# Autodesk Inventor assembly: DuoCopter - Montagem
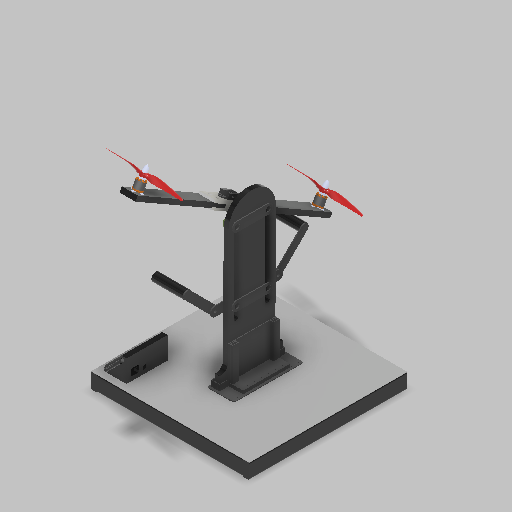
[picture p0: Inventor's stored thumbnail of the model, 512x512]
Saved by Autodesk Inventor 2025.2 (Build 292293000, 293)
## iProperties
Created: 2024-04-26
Part Number: DuoCopter - Montagem
Document SubType Name: Assembly
Designer: phmca
Author: phmca
## Documents named in this file (19)
- C:\Users\phmca\OneDrive\Área de Trabalho\GitHub\Modelos 3D\Montagem da planta\DuoCopter - Montagem.iam
- C:\Users\phmca\OneDrive\Área de Trabalho\GitHub\Modelos 3D\Montagem da planta\Chapa - aço galvanizado.ipt
- C:\Users\phmca\OneDrive\Área de Trabalho\GitHub\Modelos 3D\Montagem da planta\Painel Vertical.ipt
- C:\Users\phmca\OneDrive\Área de Trabalho\GitHub\Modelos 3D\Montagem da planta\Ripas - Base - 458 mm.ipt
- C:\Users\phmca\OneDrive\Área de Trabalho\GitHub\Modelos 3D\Montagem da planta\Ripas - Base - 500 mm.ipt
- C:\Users\phmca\OneDrive\Área de Trabalho\GitHub\Modelos 3D\Montagem da planta\Ripas - Base - 200 mm.ipt
- C:\Users\phmca\OneDrive\Área de Trabalho\GitHub\Modelos 3D\Montagem da planta\Modelos externos\Mancal de rolamento - SKF\SKF_UCFL 205.iam
- C:\Users\phmca\OneDrive\Área de Trabalho\GitHub\Modelos 3D\Montagem da planta\Junta.ipt
- C:\Users\phmca\OneDrive\Área de Trabalho\GitHub\Modelos 3D\Montagem da planta\Pás - Hastes.ipt
- C:\Users\phmca\OneDrive\Área de Trabalho\GitHub\Modelos 3D\Montagem da planta\Chapa - Aperto fixação.ipt
- C:\Users\phmca\OneDrive\Área de Trabalho\GitHub\Modelos 3D\Montagem da planta\Base - Batentes.ipt
- C:\Users\phmca\OneDrive\Área de Trabalho\GitHub\Modelos 3D\Montagem da planta\Batente limitador.ipt
- C:\Users\phmca\OneDrive\Área de Trabalho\GitHub\Modelos 3D\Montagem da planta\Base - Painel vertical.ipt
- C:\Users\phmca\OneDrive\Área de Trabalho\GitHub\Modelos 3D\Montagem da planta\Modelos externos\Motor brushless e hélices\assembly\assembly_motor.iam
- C:\Users\phmca\OneDrive\Área de Trabalho\GitHub\Modelos 3D\Montagem da planta\Case - IMU.ipt
- C:\Users\phmca\OneDrive\Área de Trabalho\GitHub\Modelos 3D\Montagem da planta\Modelos externos\Módulo MPU 6050\MPU_6050 v1.iam
- C:\Users\phmca\OneDrive\Área de Trabalho\CASE - IHM V2.ipt
- C:\Users\phmca\Downloads\nextion-3-5-hmi-nx4832t035-1.snapshot.7\Nextion 3.5 inch HMI (NX4832T035)\Nextion_3.5_HMI_NX4832T035\Nextion_3.5_HMI_NX4832T035\Nextion_3.5_HMI_NX4832T035.ipt
- C:\Users\phmca\OneDrive\Área de Trabalho\GitHub\Modelos 3D\Montagem da planta\Caneta - IHM.ipt
## Components (28 placed, 18 different names)
1. Chapa - aço galvanizado:1 — Alinhado:14, Alinhado:15, Coincidente:7, Coincidente:26, Coincidente:60, Coincidente:63
2. Painel Vertical:1 — Alinhado:9, Coincidente:3, Coincidente:5, Alinhado:13, Rotativa:1, Rotativa:2, Rotativa:4, Coincidente:13, Coincidente:16, Coincidente:27, Coincidente:31, Coincidente:36, Coincidente:37, Coincidente:46, Coincidente:61, Coincidente:62
3. Ripas - Base - 458 mm:1 — Rígida:3, Alinhado:15
4. Ripas - Base - 500 mm:1 — Rígida:2, Rígida:3, Coincidente:1, Coincidente:2
5. Ripas - Base - 500 mm:2 — Rígida:1, Alinhado:3, Alinhado:6, Alinhado:14, Coincidente:7
6. Ripas - Base - 458 mm:2 — Rígida:1, Rígida:2
7. Ripas - Base - 458 mm:3 — Alinhado:3, Coincidente:1
8. Ripas - Base - 458 mm:4 — Alinhado:6, Coincidente:2, Alinhado:9, Coincidente:3, Coincidente:4, Alinhado:11
9. Ripas - Base - 200 mm:1 — Alinhado:13
10. Ripas - Base - 200 mm:2 — Coincidente:4, Alinhado:11, Coincidente:5
11. SKF_UCFL 205:1 [sub-assembly] — Rotativa:1, Rotativa:2, Rotativa:3
12. Junta:1 — Rotativa:3, Coincidente:8, Coincidente:9, Alinhado:16, Coincidente:10, Coincidente:11, Alinhado:17, Rotativa:7, Alinhado:21
13. Pás - Hastes:1 — Coincidente:10, Coincidente:11, Alinhado:17, Coincidente:49, Tangente:1, Tangente:2
14. Pás - Hastes:2 — Coincidente:8, Coincidente:9, Alinhado:16, Coincidente:54
15. Chapa - Aperto fixação:1 — Rotativa:4, Coincidente:31
16. Base - Batentes:1 — Coincidente:13, Rotativa:5, Rotativa:6, Rotativa:8
17. Batente limitador:1 — Rotativa:5, Tangente:1, Rotativa:8, Tangente:2
18. Batente limitador:2 — Rotativa:6
19. Chapa - Aperto fixação:2 — Coincidente:16
20. Base - Painel vertical:1 — Coincidente:26, Coincidente:27, Coincidente:36, Coincidente:37, Coincidente:46
21. assembly_motor:1 [sub-assembly] — Coincidente:49
22. assembly_motor:2 [sub-assembly] — Coincidente:54
23. Case - IMU:1 — Rotativa:7, Alinhado:21, Rotativa:9
24. MPU_6050 v1:1 [sub-assembly] — Rotativa:9
25. Base - Painel vertical:3 — Coincidente:60, Coincidente:61, Coincidente:62
26. CASE - IHM V2:1 — Coincidente:63, Rotativa:10, Rotativa:11
27. Nextion_3.5_HMI_NX4832T035:1 — Rotativa:10
28. Caneta - IHM:1 — Rotativa:11
## Relationships (50: Mate 24, RevoluteJoint 11, Flush 10, WeldJoint 3, Tangent 2)
- Rígida:1 [WeldJoint]: Ripas - Base - 500 mm:2 ↔ Ripas - Base - 458 mm:2
- Rígida:2 [WeldJoint]: Ripas - Base - 500 mm:1 ↔ Ripas - Base - 458 mm:2
- Rígida:3 [WeldJoint]: Ripas - Base - 458 mm:1 ↔ Ripas - Base - 500 mm:1
- Alinhado:3 [Flush]: Ripas - Base - 500 mm:2 ↔ Ripas - Base - 458 mm:3
- Coincidente:1 [Mate]: Ripas - Base - 500 mm:1 ↔ Ripas - Base - 458 mm:3
- Alinhado:6 [Flush]: Ripas - Base - 500 mm:2 ↔ Ripas - Base - 458 mm:4
- Coincidente:2 [Mate]: Ripas - Base - 500 mm:1 ↔ Ripas - Base - 458 mm:4
- Alinhado:9 [Flush]: Painel Vertical:1 ↔ Ripas - Base - 458 mm:4
- Coincidente:3 [Mate]: Painel Vertical:1 ↔ Ripas - Base - 458 mm:4
- Coincidente:4 [Mate]: Ripas - Base - 458 mm:4 ↔ Ripas - Base - 200 mm:2
- Alinhado:11 [Flush]: Ripas - Base - 458 mm:4 ↔ Ripas - Base - 200 mm:2
- Coincidente:5 [Mate]: Painel Vertical:1 ↔ Ripas - Base - 200 mm:2
- Alinhado:13 [Flush]: Painel Vertical:1 ↔ Ripas - Base - 200 mm:1
- Alinhado:14 [Flush]: Chapa - aço galvanizado:1 ↔ Ripas - Base - 500 mm:2
- Alinhado:15 [Flush]: Chapa - aço galvanizado:1 ↔ Ripas - Base - 458 mm:1
- Coincidente:7 [Mate]: Chapa - aço galvanizado:1 ↔ Ripas - Base - 500 mm:2
- Rotativa:1 [RevoluteJoint]: Painel Vertical:1 ↔ SKF_UCFL 205:1
- Rotativa:2 [RevoluteJoint]: Painel Vertical:1 ↔ SKF_UCFL 205:1
- Rotativa:3 [RevoluteJoint]: SKF_UCFL 205:1 ↔ Junta:1
- Coincidente:8 [Mate]: Junta:1 ↔ Pás - Hastes:2
- Coincidente:9 [Mate]: Junta:1 ↔ Pás - Hastes:2
- Alinhado:16 [Flush]: Junta:1 ↔ Pás - Hastes:2
- Coincidente:10 [Mate]: Junta:1 ↔ Pás - Hastes:1
- Coincidente:11 [Mate]: Junta:1 ↔ Pás - Hastes:1
- Alinhado:17 [Flush]: Junta:1 ↔ Pás - Hastes:1
- Rotativa:4 [RevoluteJoint]: Painel Vertical:1 ↔ Chapa - Aperto fixação:1
- Coincidente:13 [Mate]: Painel Vertical:1 ↔ Base - Batentes:1
- Rotativa:5 [RevoluteJoint]: Base - Batentes:1 ↔ Batente limitador:1
- Rotativa:6 [RevoluteJoint]: Base - Batentes:1 ↔ Batente limitador:2
- Coincidente:16 [Mate]: Painel Vertical:1 ↔ Chapa - Aperto fixação:2
- Coincidente:26 [Mate]: Chapa - aço galvanizado:1 ↔ Base - Painel vertical:1
- Coincidente:27 [Mate]: Painel Vertical:1 ↔ Base - Painel vertical:1
- Coincidente:31 [Mate]: Painel Vertical:1 ↔ Chapa - Aperto fixação:1
- Coincidente:36 [Mate]: Painel Vertical:1 ↔ Base - Painel vertical:1
- Coincidente:37 [Mate]: Painel Vertical:1 ↔ Base - Painel vertical:1
- Coincidente:46 [Mate]: Painel Vertical:1 ↔ Base - Painel vertical:1
- Coincidente:49 [Mate]: Pás - Hastes:1 ↔ assembly_motor:1
- Coincidente:54 [Mate]: Pás - Hastes:2 ↔ assembly_motor:2
- Tangente:1: Pás - Hastes:1 ↔ Batente limitador:1
- Rotativa:7 [RevoluteJoint]: Junta:1 ↔ Case - IMU:1
- Alinhado:21 [Flush]: Junta:1 ↔ Case - IMU:1
- Rotativa:8 [RevoluteJoint]: Base - Batentes:1 ↔ Batente limitador:1
- Tangente:2: Pás - Hastes:1 ↔ Batente limitador:1
- Rotativa:9 [RevoluteJoint]: Case - IMU:1 ↔ MPU_6050 v1:1
- Coincidente:60 [Mate]: Chapa - aço galvanizado:1 ↔ Base - Painel vertical:3
- Coincidente:61 [Mate] (0.5 mm): Painel Vertical:1 ↔ Base - Painel vertical:3
- Coincidente:62 [Mate] (1 mm): Painel Vertical:1 ↔ Base - Painel vertical:3
- Coincidente:63 [Mate]: Chapa - aço galvanizado:1 ↔ CASE - IHM V2:1
- Rotativa:10 [RevoluteJoint]: CASE - IHM V2:1 ↔ Nextion_3.5_HMI_NX4832T035:1
- Rotativa:11 [RevoluteJoint]: CASE - IHM V2:1 ↔ Caneta - IHM:1
